# Autodesk Inventor assembly: Neo_Circle_12
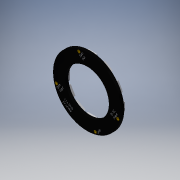
[picture p0: Inventor's stored thumbnail of the model, 180x180]
Saved by Autodesk Inventor 2017 (Build 210142000, 142)
## iProperties
Created: 2018-11-04
Part Number: Neo_Circle_12
Document SubType Name: Assembly
Designer: ludov
Author: ludov
## Documents named in this file (3)
- C:\Users\ludov\Dropbox\Electronique\Vario\Hardware\V3.00\Neo_Circle_12.iam
- C:\Users\ludov\Dropbox\Electronique\Vario\Hardware\V3.00\Neo_Cercle.ipt
- C:\Users\ludov\Dropbox\Electronique\Vario\Hardware\V3.00\Neo_Led_Complette.iam
## Components (13 placed, 2 different names)
1. Neo_Cercle:1 — Placage:1, Placage:2, Placage:3
2. Neo_Led_Complette:1 [sub-assembly] — Placage:1, Placage:2, Placage:3
3. Neo_Led_Complette:2 [sub-assembly]
4. Neo_Led_Complette:3 [sub-assembly]
5. Neo_Led_Complette:4 [sub-assembly]
6. Neo_Led_Complette:5 [sub-assembly]
7. Neo_Led_Complette:6 [sub-assembly]
8. Neo_Led_Complette:7 [sub-assembly]
9. Neo_Led_Complette:8 [sub-assembly]
10. Neo_Led_Complette:9 [sub-assembly]
11. Neo_Led_Complette:10 [sub-assembly]
12. Neo_Led_Complette:11 [sub-assembly]
13. Neo_Led_Complette:12 [sub-assembly]
## Component patterns: (12 elements, first: Neo_Led_Complette:1)
## Relationships (3: Mate 3)
- Placage:1 [Mate]: Neo_Cercle:1 ↔ Neo_Led_Complette:1
- Placage:2 [Mate] (-2.4 mm): Neo_Cercle:1 ↔ Neo_Led_Complette:1
- Placage:3 [Mate] (12.3 mm): Neo_Cercle:1 ↔ Neo_Led_Complette:1
